# Autodesk Inventor assembly: Assembly trick
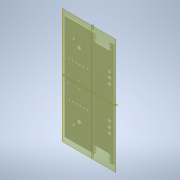
[picture p0: Inventor's stored thumbnail of the model, 180x180]
Saved by Autodesk Inventor 2022.2 (Build 262287030, 287C)
## iProperties
Created: 2022-06-15
Part Number: Assembly trick
Document SubType Name: Assembly
Designer: Andrea
Author: Andrea
## Documents named in this file (2)
- C:\Users\soffi\OneDrive\In_Row_Cultivation_Project\CAD\To_Print\Assembly trick.iam
- C:\Users\soffi\OneDrive\In_Row_Cultivation_Project\CAD\ZIP\Plate_V1.ipt
## Components (1 placed, 1 different names)
1. Plate_V1:1 — Mate:1, Mate:2, Mate:3
## Relationships (3: Mate 3)
- Mate:1: Plate_V1:1
- Mate:2: Plate_V1:1
- Mate:3: Plate_V1:1
